# Autodesk Inventor assembly: arm
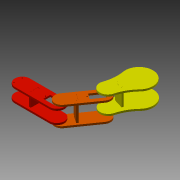
[picture p0: Inventor's stored thumbnail of the model, 180x180]
Saved by Autodesk Inventor 2013 (Build 170138000, 138)
## iProperties
Created: 2012-09-09
Part Number: arm
Document SubType Name: Assembly
Designer: frankenteddy
Author: frankenteddy
## Documents named in this file (4)
- C:\Users\frankenteddy\Desktop\oshawatt1\arm-assembled.iam
- C:\Users\frankenteddy\Desktop\oshawatt1\arm-first.iam
- C:\Users\frankenteddy\Desktop\oshawatt1\arm-second.iam
- C:\Users\frankenteddy\Desktop\oshawatt1\arm-third.iam
## Components (3 placed, 3 different names)
1. arm-first:1 [sub-assembly] — Mate:1
2. arm-second:1 [sub-assembly] — Mate:1, Mate:2
3. arm-third:1 [sub-assembly] — Mate:2
## Relationships (2: Mate 2)
- Mate:1: arm-first:1 ↔ arm-second:1
- Mate:2 (9 mm): arm-second:1 ↔ arm-third:1
